# Autodesk Inventor assembly: E3DChimera
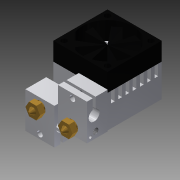
[picture p0: Inventor's stored thumbnail of the model, 180x180]
Saved by Autodesk Inventor 2015 SP1 (Build 190203100, 203)
## iProperties
Category: Hardware
Created: 2014-11-28
Part Number: E3DChimera
Document SubType Name: Assembly
Designer: Jack
Mass: 65.2728 g
Surface Area: 197.284 cm^2
Volume: 22.9553 cm^3
Density: 2.84348 g/cm^3
Vendor: E3D
Catalog Web Link: http://e3d-online.com/Chimera
Author: Jack
Title: E3D Chimera
## Documents named in this file (7)
- C:\Users\Jack\ownCloud\Projects\CrossBot\InventorModel\HotEnds\E3DChimera\E3DChimera.iam
- C:\Users\Jack\ownCloud\Projects\CrossBot\InventorModel\HotEnds\E3DChimera\E3DBowdenInsert.ipt
- C:\Users\Jack\ownCloud\Projects\CrossBot\InventorModel\HotEnds\E3DChimera\ChimeraHeatsink.ipt
- C:\Users\Jack\ownCloud\Projects\CrossBot\InventorModel\HotEnds\E3DChimera\Fan30mm.ipt
- C:\Users\Jack\ownCloud\Projects\CrossBot\InventorModel\HotEnds\E3DChimera\ChimeraHeatBreak.ipt
- C:\Users\Jack\ownCloud\Projects\CrossBot\InventorModel\HotEnds\E3DChimera\ChimeraHeatBlock.ipt
- C:\Users\Jack\ownCloud\Projects\CrossBot\InventorModel\HotEnds\E3DChimera\ChimeraNozzle.4.ipt
## Components (10 placed, 6 different names)
1. E3DBowdenInsert:1 — Mate:4, Mate:6
2. E3DBowdenInsert:2 — Mate:5, Mate:7
3. ChimeraHeatsink:1 — Mate:1, Mate:2, Mate:3, Mate:4, Mate:5, Mate:6, Mate:7, Mate:8, Flush:1, Flush:2, Mate:9, Mate:10, Mate:11, Mate:12, Angle:2
4. Fan30mm:1 — Mate:8, Flush:1, Flush:2
5. ChimeraHeatBreak:1 — Mate:9, Mate:11, Mate:14, Mate:17, Flush:4
6. ChimeraHeatBreak:2 — Mate:10, Mate:12, Mate:13, Mate:18
7. ChimeraHeatBlock:1 — Mate:13, Mate:16, Angle:1, Flush:3
8. ChimeraHeatBlock:2 — Mate:14, Mate:15, Angle:1, Angle:2, Flush:3, Flush:4
9. ChimeraNozzle.4:1 — Mate:15, Mate:17
10. ChimeraNozzle.4:2 — Mate:16, Mate:18
## Relationships (24: Mate 18, Flush 4, Angle 2)
- Mate:1: ChimeraHeatsink:1
- Mate:2: ChimeraHeatsink:1
- Mate:3: ChimeraHeatsink:1
- Mate:4: E3DBowdenInsert:1 ↔ ChimeraHeatsink:1
- Mate:5: E3DBowdenInsert:2 ↔ ChimeraHeatsink:1
- Mate:6: E3DBowdenInsert:1 ↔ ChimeraHeatsink:1
- Mate:7: E3DBowdenInsert:2 ↔ ChimeraHeatsink:1
- Mate:8: ChimeraHeatsink:1 ↔ Fan30mm:1
- Flush:1: ChimeraHeatsink:1 ↔ Fan30mm:1
- Flush:2: ChimeraHeatsink:1 ↔ Fan30mm:1
- Mate:9: ChimeraHeatsink:1 ↔ ChimeraHeatBreak:1
- Mate:10: ChimeraHeatsink:1 ↔ ChimeraHeatBreak:2
- Mate:11: ChimeraHeatsink:1 ↔ ChimeraHeatBreak:1
- Mate:12: ChimeraHeatsink:1 ↔ ChimeraHeatBreak:2
- Mate:13: ChimeraHeatBreak:2 ↔ ChimeraHeatBlock:1
- Mate:14: ChimeraHeatBreak:1 ↔ ChimeraHeatBlock:2
- Mate:15: ChimeraHeatBlock:2 ↔ ChimeraNozzle.4:1
- Mate:16: ChimeraHeatBlock:1 ↔ ChimeraNozzle.4:2
- Mate:17: ChimeraHeatBreak:1 ↔ ChimeraNozzle.4:1
- Mate:18: ChimeraHeatBreak:2 ↔ ChimeraNozzle.4:2
- Angle:1 (0 deg): ChimeraHeatBlock:1 ↔ ChimeraHeatBlock:2
- Angle:2 (0 deg): ChimeraHeatsink:1 ↔ ChimeraHeatBlock:2
- Flush:3: ChimeraHeatBlock:1 ↔ ChimeraHeatBlock:2
- Flush:4: ChimeraHeatBreak:1 ↔ ChimeraHeatBlock:2
